# Autodesk Inventor assembly: Final_Reduccion
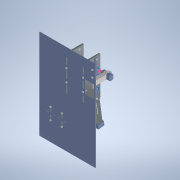
[picture p0: Inventor's stored thumbnail of the model, 180x180]
Saved by Autodesk Inventor 2022 (Build 260153000, 153)
## iProperties
Created: 2022-03-13
Part Number: Final_Reduccion
Document SubType Name: Assembly
Designer: katha
Author: katha
## Documents named in this file (24)
- C:\Users\katha\OneDrive\Escritorio\Mini_Proyecto_Diseno\Diseno_18012\Modelo_MPD\Final_Reduccion.iam
- C:\Users\katha\OneDrive\Escritorio\Mini_Proyecto_Diseno\Diseno_18012\Modelo_MPD\eje1_n.ipt
- C:\Users\katha\OneDrive\Escritorio\Mini_Proyecto_Diseno\Diseno_18012\Modelo_MPD\eje2_n.ipt
- C:\Users\katha\OneDrive\Escritorio\Mini_Proyecto_Diseno\Diseno_18012\Modelo_MPD\eje3_n.ipt
- C:\Users\katha\OneDrive\Escritorio\Mini_Proyecto_Diseno\Diseno_18012\Modelo_MPD\engranaje40.ipt
- C:\Users\katha\OneDrive\Escritorio\Mini_Proyecto_Diseno\Diseno_18012\Modelo_MPD\engranaje10.ipt
- C:\Users\katha\OneDrive\Escritorio\Mini_Proyecto_Diseno\Diseno_18012\Modelo_MPD\hombro_nuevo.ipt
- C:\Users\katha\OneDrive\Escritorio\Mini_Proyecto_Diseno\Diseno_18012\Modelo_MPD\eje4_n.ipt
- C:\Users\katha\OneDrive\Escritorio\Mini_Proyecto_Diseno\Diseno_18012\Modelo_MPD\Base_proyecto.ipt
- C:\Users\katha\OneDrive\Escritorio\Mini_Proyecto_Diseno\Diseno_18012\Modelo_MPD\caja_2_Lateral.ipt
- C:\Users\katha\OneDrive\Escritorio\Mini_Proyecto_Diseno\Diseno_18012\Modelo_MPD\Rodamiento_Ejes.ipt
- C:\Users\katha\OneDrive\Escritorio\Mini_Proyecto_Diseno\Diseno_18012\Modelo_MPD\Acople_Motor_.ipt
- C:\Users\katha\OneDrive\Escritorio\Mini_Proyecto_Diseno\Diseno_18012\Modelo_MPD\sujetador_motor.ipt
- C:\Users\katha\OneDrive\Escritorio\Mini_Proyecto_Diseno\Diseno_18012\Modelo_MPD\motor_12v.ipt
- C:\Users\katha\OneDrive\Escritorio\Mini_Proyecto_Diseno\Diseno_18012\Modelo_MPD\Base.ipt
- C:\Users\katha\OneDrive\Escritorio\Mini_Proyecto_Diseno\Diseno_18012\Modelo_MPD\Acople_TransPot.ipt
- C:\Users\katha\OneDrive\Escritorio\Mini_Proyecto_Diseno\Diseno_18012\Modelo_MPD\Base_Soporte.ipt
- C:\Users\katha\OneDrive\Escritorio\Mini_Proyecto_Diseno\Diseno_18012\Modelo_MPD\Carcasa_Tope.ipt
- C:\Users\katha\OneDrive\Escritorio\Mini_Proyecto_Diseno\Diseno_18012\Modelo_MPD\Carril.iam
- C:\Users\katha\OneDrive\Escritorio\Mini_Proyecto_Diseno\Diseno_18012\Modelo_MPD\Eslabon_TransPot.ipt
- C:\Users\katha\OneDrive\Escritorio\Mini_Proyecto_Diseno\Diseno_18012\Modelo_MPD\M4_long.ipt
- C:\Users\katha\OneDrive\Escritorio\Mini_Proyecto_Diseno\Diseno_18012\Modelo_MPD\M4_short.ipt
- C:\Users\katha\OneDrive\Escritorio\Mini_Proyecto_Diseno\Diseno_18012\Modelo_MPD\M4_tuerca.ipt
- C:\Users\katha\OneDrive\Escritorio\Mini_Proyecto_Diseno\Diseno_18012\Modelo_MPD\rodamiento_carril.ipt
## Components (70 placed, 23 different names)
1. eje1_n:1 — Mate:1, Mate:2, Mate:3, Mate:4, Mate:5, Flush:1, Mate:45, Mate:46, Flush:21, Mate:54, Mate:61, Mate:62, Mate:63
2. eje2_n:1 — Flush:1, Mate:8, Mate:9, Mate:10, Flush:4, Mate:12, Mate:13, Mate:43, Mate:44, Mate:53
3. engranaje40:1 — Mate:4, Mate:5, Mate:6
4. hombro_nuevo:1 — Mate:1, Mate:2, Mate:3, Mate:6
5. hombro_nuevo:2 — Mate:8, Mate:9, Mate:10, Flush:2, Flush:3, Mate:11
6. engranaje10:1 — Flush:2, Flush:3, Mate:11, Mate:14
7. eje3_n:1 — Flush:4, Mate:15, Mate:16, Mate:17, Mate:19, Mate:20, Flush:7, Mate:41, Flush:20, Mate:42, Mate:52
8. engranaje40:2 — Mate:12, Mate:13, Mate:14
9. hombro_nuevo:3 — Mate:15, Mate:16, Mate:17, Mate:21
10. engranaje10:2 — Flush:5, Flush:6, Mate:18, Mate:19, Mate:20, Mate:21
11. engranaje40:3 — Flush:5, Flush:6, Mate:18
12. eje4_n:1 — Mate:22, Mate:23, Mate:24, Flush:7, Mate:25, Mate:26, Mate:39, Flush:19, Mate:40, Mate:47, Mate:48
13. hombro_nuevo:4 — Mate:22, Mate:23, Mate:24, Mate:27
14. engranaje10:3 — Mate:25, Mate:26, Mate:27
15. Base_proyecto:1 — Mate:28, Mate:29, Flush:8, Mate:30, Flush:22, Mate:55, Mate:56, Flush:23, Mate:57, Mate:58, Mate:59, Mate:60, Mate:77, Mate:78, Mate:79, Mate:80, Mate:81, Mate:82, Mate:83, Mate:84, Mate:85, Mate:86, Mate:87, Mate:88, Mate:89, Mate:90, Mate:91, Mate:92, Mate:99, Mate:100
16. caja_2_Lateral:1 — Mate:28, Mate:29, Flush:8, Flush:9, Flush:10, Mate:31, Mate:32, Mate:33, Mate:34, Flush:15, Flush:16, Flush:17, Flush:18, Mate:64, Mate:65, Mate:66, Mate:121, Mate:123, Mate:133
17. caja_2_Lateral:2 — Flush:9, Flush:10, Mate:30, Mate:35, Mate:36, Mate:37, Mate:38, Flush:11, Flush:12, Flush:13, Flush:14, Mate:67, Mate:68, Mate:69, Mate:114, Mate:129, Mate:130
18. Rodamiento_Ejes:1 — Mate:31, Flush:15, Flush:19, Mate:40
19. Rodamiento_Ejes:2 — Mate:32, Flush:16, Mate:41, Flush:20, Mate:42
20. Rodamiento_Ejes:3 — Mate:33, Flush:17, Mate:43, Mate:44
21. Rodamiento_Ejes:4 — Mate:34, Flush:18, Mate:45, Mate:46
22. Rodamiento_Ejes:5 — Mate:38, Flush:11, Flush:21, Mate:54
23. Rodamiento_Ejes:6 — Mate:37, Flush:12, Mate:53
24. Rodamiento_Ejes:7 — Mate:36, Flush:13, Mate:52
25. Rodamiento_Ejes:8 — Mate:35, Flush:14, Mate:39
26. Acople_Motor_:1 — Mate:47, Mate:48, Mate:49, Mate:50
27. sujetador_motor:1 — Flush:22, Mate:51, Mate:97, Mate:98, Mate:112, Mate:113
28. motor_12v:1 — Mate:49, Mate:50, Mate:51
29. Base:1 — Mate:57, Mate:58, Flush:24, Flush:25, Mate:72, Mate:75, Mate:76, Mate:115
30. Base:2 — Mate:55, Mate:56, Flush:23, Flush:24, Mate:119
31. Acople_TransPot:1 — Mate:61, Mate:62, Mate:63, Mate:70, Mate:71, Mate:118
32. Base_Soporte:1 — Mate:59, Mate:60, Flush:25
33. Carcasa_Tope:1 — Mate:64, Mate:65, Mate:66, Mate:126
34. Carcasa_Tope:2 — Mate:67, Mate:68, Mate:69, Mate:120, Mate:122, Mate:124, Mate:125
35. Carril:1 [sub-assembly] — Mate:72, Mate:73, Mate:74, Mate:93, Mate:94, Flush:26
36. Eslabon_TransPot:1 — Mate:70, Mate:71, Mate:73, Mate:74, Mate:95, Mate:96
37. M4_long:1 — Mate:75, Mate:76, Mate:101, Mate:117
38. M4_short:1 — Mate:77, Mate:92, Mate:102
39. M4_short:2 — Mate:80, Mate:86, Mate:104
40. M4_short:3 — Mate:78, Mate:91, Mate:103
41. M4_short:4 — Mate:79, Mate:85, Mate:105
42. M4_short:5 — Mate:81, Mate:90, Mate:106
43. M4_short:6 — Mate:84, Mate:87, Mate:108
44. M4_short:7 — Mate:82, Mate:89, Mate:107
45. M4_short:8 — Mate:83, Mate:88, Mate:111
46. M4_short:10 — Mate:97, Mate:100, Mate:110
47. M4_short:11 — Mate:98, Mate:99, Mate:109
48. M4_short:12 — Mate:93, Mate:94
49. M4_short:13 — Mate:95, Mate:96, Mate:116
50. M4_tuerca:1 — Mate:102, Mate:115, Flush:30, Flush:31
51. M4_tuerca:2 — Mate:103, Flush:30
52. M4_tuerca:3 — Mate:104, Flush:32
53. M4_tuerca:4 — Mate:105, Flush:31, Flush:32
54. M4_tuerca:5 — Mate:107, Flush:29
55. M4_tuerca:6 — Mate:111, Flush:27
56. M4_tuerca:7 — Mate:106, Flush:28
57. M4_tuerca:8 — Mate:108, Mate:114, Flush:27, Flush:28, Flush:29
58. M4_tuerca:9 — Mate:109, Mate:112
59. M4_tuerca:10 — Mate:110, Mate:113
60. M4_tuerca:13 — Mate:117, Mate:119
61. M4_tuerca:14 — Mate:116, Mate:118
62. rodamiento_carril:1 — Mate:101, Flush:26
63. M4_short:14 — Mate:120, Mate:125, Mate:128
64. M4_short:15 — Mate:122, Mate:124, Mate:127
65. M4_short:16 — Mate:121, Mate:126, Flush:33, Mate:131
66. M4_short:17 — Mate:123, Flush:33, Mate:132
67. M4_tuerca:16 — Mate:131, Mate:133, Flush:34
68. M4_tuerca:17 — Mate:132, Flush:34
69. M4_tuerca:18 — Mate:127, Mate:130
70. M4_tuerca:19 — Mate:128, Mate:129
## Relationships (166: Mate 132, Flush 34)
- Mate:1 (0.45 mm): eje1_n:1 ↔ hombro_nuevo:1
- Mate:2 (0.45 mm): eje1_n:1 ↔ hombro_nuevo:1
- Mate:3: eje1_n:1 ↔ hombro_nuevo:1
- Mate:4 (0.45 mm): eje1_n:1 ↔ engranaje40:1
- Mate:5 (0.45 mm): eje1_n:1 ↔ engranaje40:1
- Mate:6: engranaje40:1 ↔ hombro_nuevo:1
- Flush:1: eje1_n:1 ↔ eje2_n:1
- Mate:8 (0.45 mm): eje2_n:1 ↔ hombro_nuevo:2
- Mate:9 (0.45 mm): eje2_n:1 ↔ hombro_nuevo:2
- Mate:10: eje2_n:1 ↔ hombro_nuevo:2
- Flush:2: hombro_nuevo:2 ↔ engranaje10:1
- Flush:3: hombro_nuevo:2 ↔ engranaje10:1
- Mate:11: hombro_nuevo:2 ↔ engranaje10:1
- Flush:4: eje2_n:1 ↔ eje3_n:1
- Mate:12 (0.45 mm): eje2_n:1 ↔ engranaje40:2
- Mate:13 (0.45 mm): eje2_n:1 ↔ engranaje40:2
- Mate:14: engranaje10:1 ↔ engranaje40:2
- Mate:15 (0.45 mm): eje3_n:1 ↔ hombro_nuevo:3
- Mate:16 (0.45 mm): eje3_n:1 ↔ hombro_nuevo:3
- Mate:17: eje3_n:1 ↔ hombro_nuevo:3
- Flush:5: engranaje10:2 ↔ engranaje40:3
- Flush:6: engranaje10:2 ↔ engranaje40:3
- Mate:18: engranaje10:2 ↔ engranaje40:3
- Mate:19 (0.45 mm): eje3_n:1 ↔ engranaje10:2
- Mate:20 (0.45 mm): eje3_n:1 ↔ engranaje10:2
- Mate:21: hombro_nuevo:3 ↔ engranaje10:2
- Mate:22 (0.45 mm): eje4_n:1 ↔ hombro_nuevo:4
- Mate:23 (0.45 mm): eje4_n:1 ↔ hombro_nuevo:4
- Mate:24: eje4_n:1 ↔ hombro_nuevo:4
- Flush:7: eje3_n:1 ↔ eje4_n:1
- Mate:25 (0.45 mm): eje4_n:1 ↔ engranaje10:3
- Mate:26 (0.45 mm): eje4_n:1 ↔ engranaje10:3
- Mate:27: hombro_nuevo:4 ↔ engranaje10:3
- Mate:28: Base_proyecto:1 ↔ caja_2_Lateral:1
- Mate:29: Base_proyecto:1 ↔ caja_2_Lateral:1
- Flush:8: Base_proyecto:1 ↔ caja_2_Lateral:1
- Flush:9: caja_2_Lateral:1 ↔ caja_2_Lateral:2
- Flush:10: caja_2_Lateral:1 ↔ caja_2_Lateral:2
- Mate:30: Base_proyecto:1 ↔ caja_2_Lateral:2
- Mate:31: caja_2_Lateral:1 ↔ Rodamiento_Ejes:1
- Mate:32: caja_2_Lateral:1 ↔ Rodamiento_Ejes:2
- Mate:33: caja_2_Lateral:1 ↔ Rodamiento_Ejes:3
- Mate:34: caja_2_Lateral:1 ↔ Rodamiento_Ejes:4
- Mate:35: caja_2_Lateral:2 ↔ Rodamiento_Ejes:8
- Mate:36: caja_2_Lateral:2 ↔ Rodamiento_Ejes:7
- Mate:37: caja_2_Lateral:2 ↔ Rodamiento_Ejes:6
- Mate:38: caja_2_Lateral:2 ↔ Rodamiento_Ejes:5
- Flush:11 (0.1 mm): caja_2_Lateral:2 ↔ Rodamiento_Ejes:5
- Flush:12 (0.1 mm): caja_2_Lateral:2 ↔ Rodamiento_Ejes:6
- Flush:13 (-0.1 mm): caja_2_Lateral:2 ↔ Rodamiento_Ejes:7
- Flush:14 (-0.1 mm): caja_2_Lateral:2 ↔ Rodamiento_Ejes:8
- Flush:15 (0.1 mm): caja_2_Lateral:1 ↔ Rodamiento_Ejes:1
- Flush:16 (0.1 mm): caja_2_Lateral:1 ↔ Rodamiento_Ejes:2
- Flush:17 (0.1 mm): caja_2_Lateral:1 ↔ Rodamiento_Ejes:3
- Flush:18 (0.1 mm): caja_2_Lateral:1 ↔ Rodamiento_Ejes:4
- Mate:39 (0.45 mm): eje4_n:1 ↔ Rodamiento_Ejes:8
- Flush:19: eje4_n:1 ↔ Rodamiento_Ejes:1
- Mate:40 (0.45 mm): eje4_n:1 ↔ Rodamiento_Ejes:1
- Mate:41 (0.45 mm): eje3_n:1 ↔ Rodamiento_Ejes:2
- Flush:20: eje3_n:1 ↔ Rodamiento_Ejes:2
- Mate:42 (0.45 mm): eje3_n:1 ↔ Rodamiento_Ejes:2
- Mate:43 (0.45 mm): eje2_n:1 ↔ Rodamiento_Ejes:3
- Mate:44 (0.45 mm): eje2_n:1 ↔ Rodamiento_Ejes:3
- Mate:45 (0.45 mm): eje1_n:1 ↔ Rodamiento_Ejes:4
- Mate:46 (0.45 mm): eje1_n:1 ↔ Rodamiento_Ejes:4
- Flush:21: eje1_n:1 ↔ Rodamiento_Ejes:5
- Mate:47: eje4_n:1 ↔ Acople_Motor_:1
- Mate:48 (0.4 mm): eje4_n:1 ↔ Acople_Motor_:1
- Flush:22: Base_proyecto:1 ↔ sujetador_motor:1
- Mate:49: Acople_Motor_:1 ↔ motor_12v:1
- Mate:50 (1 mm): Acople_Motor_:1 ↔ motor_12v:1
- Mate:51 (0.2 mm): sujetador_motor:1 ↔ motor_12v:1
- Mate:52 (0.45 mm): eje3_n:1 ↔ Rodamiento_Ejes:7
- Mate:53 (0.45 mm): eje2_n:1 ↔ Rodamiento_Ejes:6
- Mate:54 (0.45 mm): eje1_n:1 ↔ Rodamiento_Ejes:5
- Mate:55: Base_proyecto:1 ↔ Base:2
- Mate:56: Base_proyecto:1 ↔ Base:2
- Flush:23: Base_proyecto:1 ↔ Base:2
- Mate:57: Base_proyecto:1 ↔ Base:1
- Mate:58: Base_proyecto:1 ↔ Base:1
- Flush:24: Base:1 ↔ Base:2
- Mate:59: Base_proyecto:1 ↔ Base_Soporte:1
- Mate:60: Base_proyecto:1 ↔ Base_Soporte:1
- Flush:25: Base:1 ↔ Base_Soporte:1
- Mate:61: eje1_n:1 ↔ Acople_TransPot:1
- Mate:62 (0.4 mm): eje1_n:1 ↔ Acople_TransPot:1
- Mate:63 (0.4 mm): eje1_n:1 ↔ Acople_TransPot:1
- Mate:64: caja_2_Lateral:1 ↔ Carcasa_Tope:1
- Mate:65: caja_2_Lateral:1 ↔ Carcasa_Tope:1
- Mate:66: caja_2_Lateral:1 ↔ Carcasa_Tope:1
- Mate:67: caja_2_Lateral:2 ↔ Carcasa_Tope:2
- Mate:68: caja_2_Lateral:2 ↔ Carcasa_Tope:2
- Mate:69: caja_2_Lateral:2 ↔ Carcasa_Tope:2
- Mate:70: Acople_TransPot:1 ↔ Eslabon_TransPot:1
- Mate:71: Acople_TransPot:1 ↔ Eslabon_TransPot:1
- Mate:72: Base:1 ↔ Carril:1
- Mate:73: Carril:1 ↔ Eslabon_TransPot:1
- Mate:74: Carril:1 ↔ Eslabon_TransPot:1
- Mate:75: Base:1 ↔ M4_long:1
- Mate:76: Base:1 ↔ M4_long:1
- Mate:77: Base_proyecto:1 ↔ M4_short:1
- Mate:78: Base_proyecto:1 ↔ M4_short:3
- Mate:79: Base_proyecto:1 ↔ M4_short:4
- Mate:80: Base_proyecto:1 ↔ M4_short:2
- Mate:81: Base_proyecto:1 ↔ M4_short:5
- Mate:82: Base_proyecto:1 ↔ M4_short:7
- Mate:83: Base_proyecto:1 ↔ M4_short:8
- Mate:84: Base_proyecto:1 ↔ M4_short:6
- Mate:85: Base_proyecto:1 ↔ M4_short:4
- Mate:86: Base_proyecto:1 ↔ M4_short:2
- Mate:87: Base_proyecto:1 ↔ M4_short:6
- Mate:88: Base_proyecto:1 ↔ M4_short:8
- Mate:89: Base_proyecto:1 ↔ M4_short:7
- Mate:90: Base_proyecto:1 ↔ M4_short:5
- Mate:91: Base_proyecto:1 ↔ M4_short:3
- Mate:92: Base_proyecto:1 ↔ M4_short:1
- Mate:93: Carril:1 ↔ M4_short:12
- Mate:94: Carril:1 ↔ M4_short:12
- Mate:95: Eslabon_TransPot:1 ↔ M4_short:13
- Mate:96: Eslabon_TransPot:1 ↔ M4_short:13
- Mate:97: sujetador_motor:1 ↔ M4_short:10
- Mate:98: sujetador_motor:1 ↔ M4_short:11
- Mate:99: Base_proyecto:1 ↔ M4_short:11
- Mate:100: Base_proyecto:1 ↔ M4_short:10
- Mate:101: M4_long:1 ↔ rodamiento_carril:1
- Flush:26: Carril:1 ↔ rodamiento_carril:1
- Mate:102: M4_short:1 ↔ M4_tuerca:1
- Mate:103: M4_short:3 ↔ M4_tuerca:2
- Mate:104: M4_short:2 ↔ M4_tuerca:3
- Mate:105: M4_short:4 ↔ M4_tuerca:4
- Mate:106: M4_short:5 ↔ M4_tuerca:7
- Mate:107: M4_short:7 ↔ M4_tuerca:5
- Mate:108: M4_short:6 ↔ M4_tuerca:8
- Mate:109: M4_short:11 ↔ M4_tuerca:9
- Mate:110: M4_short:10 ↔ M4_tuerca:10
- Mate:111: M4_short:8 ↔ M4_tuerca:6
- Mate:112: sujetador_motor:1 ↔ M4_tuerca:9
- Mate:113: sujetador_motor:1 ↔ M4_tuerca:10
- Mate:114: caja_2_Lateral:2 ↔ M4_tuerca:8
- Flush:27: M4_tuerca:6 ↔ M4_tuerca:8
- Flush:28: M4_tuerca:7 ↔ M4_tuerca:8
- Flush:29: M4_tuerca:5 ↔ M4_tuerca:8
- Mate:115: Base:1 ↔ M4_tuerca:1
- Flush:30: M4_tuerca:1 ↔ M4_tuerca:2
- Flush:31: M4_tuerca:1 ↔ M4_tuerca:4
- Flush:32: M4_tuerca:3 ↔ M4_tuerca:4
- Mate:116: M4_short:13 ↔ M4_tuerca:14
- Mate:117: M4_long:1 ↔ M4_tuerca:13
- Mate:118: Acople_TransPot:1 ↔ M4_tuerca:14
- Mate:119: Base:2 ↔ M4_tuerca:13
- Mate:120: Carcasa_Tope:2 ↔ M4_short:14
- Mate:121: caja_2_Lateral:1 ↔ M4_short:16
- Mate:122: Carcasa_Tope:2 ↔ M4_short:15
- Mate:123: caja_2_Lateral:1 ↔ M4_short:17
- Mate:124: Carcasa_Tope:2 ↔ M4_short:15
- Mate:125: Carcasa_Tope:2 ↔ M4_short:14
- Mate:126: Carcasa_Tope:1 ↔ M4_short:16
- Flush:33: M4_short:16 ↔ M4_short:17
- Mate:127: M4_short:15 ↔ M4_tuerca:18
- Mate:128: M4_short:14 ↔ M4_tuerca:19
- Mate:129: caja_2_Lateral:2 ↔ M4_tuerca:19
- Mate:130: caja_2_Lateral:2 ↔ M4_tuerca:18
- Mate:131: M4_short:16 ↔ M4_tuerca:16
- Mate:132: M4_short:17 ↔ M4_tuerca:17
- Mate:133: caja_2_Lateral:1 ↔ M4_tuerca:16
- Flush:34: M4_tuerca:16 ↔ M4_tuerca:17
